# Autodesk Inventor assembly: legg_assembly
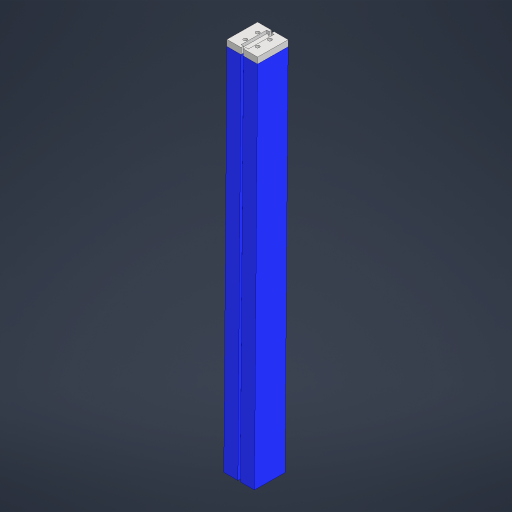
[picture p0: Inventor's stored thumbnail of the model, 512x512]
Saved by Autodesk Inventor 2024 (Build 280153000, 153)
## iProperties
Created: 2023-05-23
Part Number: legg_assembly
Document SubType Name: Assembly
Designer: aasmu
Author: aasmu
## Documents named in this file (3)
- C:\Users\aasmu\Documents\standing_desk\legg_assembly.iam
- C:\Users\aasmu\Documents\standing_desk\1_inner_leg.ipt
- C:\Users\aasmu\Documents\standing_desk\2_inner_leg_top_plate.ipt
## Components (2 placed, 2 different names)
1. 1_inner_leg:1 — Rigid:1
2. 2_inner_leg_top_plate:1 — Rigid:1
## Relationships (1: WeldJoint 1)
- Rigid:1 [WeldJoint]: 1_inner_leg:1 ↔ 2_inner_leg_top_plate:1
